# Autodesk Inventor assembly: Frame0001
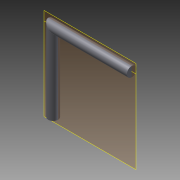
[picture p0: Inventor's stored thumbnail of the model, 180x180]
Saved by Autodesk Inventor 2013 (Build 170138000, 138)
## iProperties
Created: 2013-01-06
Part Number: Frame0001
Document SubType Name: Assembly
Designer: Phillip
_FrameDoc: Frame Assembly
_Version: 15.0.0
Author: Phillip
## Documents named in this file (6)
- E:\Data Folder\FIRST 2013\FIRST KOP\FIRST Arena 2013\Pyramid\GE-13020\Frame\Frame0001.iam
- E:\Data Folder\FIRST 2013\FIRST KOP\FIRST Arena 2013\Pyramid\GE-13020\Frame\Skeleton0001.ipt
- E:\Data Folder\FIRST 2013\FIRST KOP\FIRST Arena 2013\Pyramid\GE-13020\Frame\ANSI 1 1_2 00000001.ipt
- ANSI 1 1_2 00000001.ipt
- E:\Data Folder\FIRST 2013\FIRST KOP\FIRST Arena 2013\Pyramid\GE-13020\Frame\ANSI 1 1_2 00000002.ipt
- ANSI 1 1_2 00000002.ipt
## Components (3 placed, 3 different names)
1. Frame Reference Model
2. ANSI 1 1_2 00000001:1
3. ANSI 1 1_2 00000002:1 — Mate:1
## Relationships (3: Mate 2, Angle 1)
- Mate:1: ANSI 1 1_2 00000002:1
- Mate:2
- Angle:1 (0 deg)
